# Autodesk Inventor assembly: !Robot Assembly
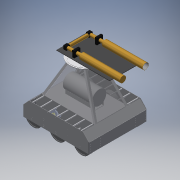
[picture p0: Inventor's stored thumbnail of the model, 180x180]
Saved by Autodesk Inventor 2016 (Build 200138000, 138)
## iProperties
Created: 2018-05-05
Part Number: !Robot Assembly
Document SubType Name: Assembly
Designer: Kade
Mass: 22226.7 g
Surface Area: 76458 cm^2
Volume: 19766 cm^3
Density: 1.1245 g/cm^3
Author: Kade
## Documents named in this file (4)
- F:\Robotics\Off Season\Blannon\!Robot Assembly.iam
- F:\Robotics\Off Season\Blannon\DT Assembly.iam
- F:\Robotics\Off Season\Blannon\Pannels Assembly V2.iam
- F:\Robotics\Off Season\Blannon\Cannon.iam
## Components (3 placed, 3 different names)
1. DT Assembly:1 [sub-assembly] — Mate:19, Mate:20, Mate:21, Mate:22, Flush:25
2. Pannels Assembly V2:1 [sub-assembly] — Mate:22, Flush:25, Angle:1, Mate:23, Flush:26, Flush:27
3. Cannon:1 [sub-assembly] — Mate:23, Flush:26, Flush:27
## Relationships (9: Mate 5, Flush 3, Angle 1)
- Mate:19: DT Assembly:1
- Mate:20: DT Assembly:1
- Mate:21: DT Assembly:1
- Mate:22: DT Assembly:1 ↔ Pannels Assembly V2:1
- Flush:25 (304.8 mm): DT Assembly:1 ↔ Pannels Assembly V2:1
- Angle:1 (180 deg): Pannels Assembly V2:1
- Mate:23: Pannels Assembly V2:1 ↔ Cannon:1
- Flush:26: Pannels Assembly V2:1 ↔ Cannon:1
- Flush:27: Pannels Assembly V2:1 ↔ Cannon:1
